# Autodesk Inventor assembly: Ensemble tout
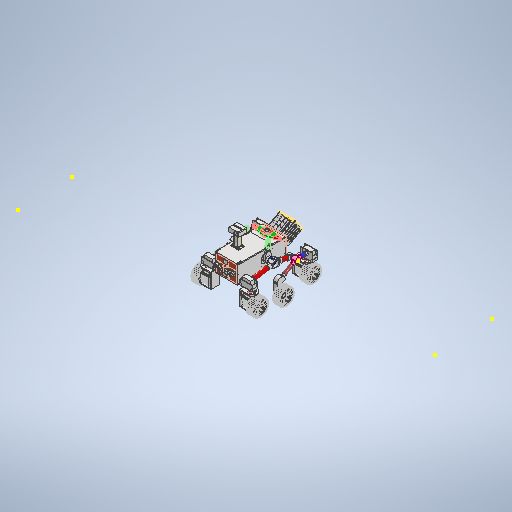
[picture p0: Inventor's stored thumbnail of the model, 512x512]
Saved by Autodesk Inventor 2026.2 (Build 302298010, 298A)
## iProperties
Created: 2026-03-16
Part Number: Ensemble tout
Document SubType Name: Assembly
Designer: genon
Author: genon
## Documents named in this file (36)
- C:\Users\genon\Documents\Henallux Passerelle\Projet de conception\Cassini T-X\Inventor\Ensemble tout.iam
- C:\Users\genon\Documents\Henallux Passerelle\Projet de conception\Cassini T-X\Inventor\Ensemble_Boite_chassis.iam
- C:\Users\genon\Documents\Henallux Passerelle\Projet de conception\Cassini T-X\Inventor\Suspension\Ensemble_Relier_suspension.iam
- C:\Users\genon\Documents\Henallux Passerelle\Projet de conception\Cassini T-X\Inventor\Suspension\tube vers bogie.ipt
- C:\Users\genon\Documents\Henallux Passerelle\Projet de conception\Cassini T-X\Inventor\Suspension\bielle sup.ipt
- C:\Users\genon\Documents\Henallux Passerelle\Projet de conception\Cassini T-X\Inventor\Suspension\bielle côté 0.ipt
- C:\Users\genon\Documents\Henallux Passerelle\Projet de conception\Cassini T-X\Inventor\Suspension\bièlle côté.ipt
- C:\Users\genon\Documents\Henallux Passerelle\Projet de conception\Cassini T-X\Inventor\Suspension\Rolling v2.ipt
- C:\Users\genon\Documents\Henallux Passerelle\Projet de conception\Cassini T-X\Inventor\Suspension\bielle côté 2.ipt
- C:\Users\genon\Documents\Henallux Passerelle\Projet de conception\Cassini T-X\Inventor\Suspension\bielle côté 3.ipt
- C:\Users\genon\Documents\Henallux Passerelle\Projet de conception\Cassini T-X\Inventor\Suspension\tubelong_rocker.ipt
- C:\Users\genon\Documents\Henallux Passerelle\Projet de conception\Cassini T-X\Inventor\Suspension\Attache servomoteur.ipt
- C:\Users\genon\Documents\Henallux Passerelle\Projet de conception\Cassini T-X\Inventor\Suspension\bielle rocker.ipt
- C:\Users\genon\Documents\Henallux Passerelle\Projet de conception\Cassini T-X\Inventor\Suspension\bielle rocker2.ipt
- C:\Users\genon\Documents\Henallux Passerelle\Projet de conception\Cassini T-X\Inventor\Suspension\tube des bogies.ipt
- C:\Users\genon\Documents\Henallux Passerelle\Projet de conception\Cassini T-X\Inventor\Suspension\Attache servomoteur_bogie.ipt
- C:\Users\genon\Documents\Henallux Passerelle\Projet de conception\Cassini T-X\Inventor\Composants\Stepper Motor\Stepper Motor\Stepper Motor.ipt
- C:\Users\genon\Documents\Henallux Passerelle\Projet de conception\Cassini T-X\Inventor\Suspension\roulement 22mm.ipt
- C:\Users\genon\Documents\Henallux Passerelle\Projet de conception\Cassini T-X\Inventor\Suspension\Roue.ipt
- C:\Users\genon\Documents\Henallux Passerelle\Projet de conception\Cassini T-X\Inventor\Suspension\Roue libre.ipt
- C:\Users\genon\Documents\Henallux Passerelle\Projet de conception\Cassini T-X\Inventor\Suspension\bielle roue milieu autre côté.ipt
- C:\Users\genon\Documents\Henallux Passerelle\Projet de conception\Cassini T-X\Inventor\Composants\US HC-SR04.ipt
- C:\Users\genon\Documents\Henallux Passerelle\Projet de conception\Cassini T-X\Inventor\Composants\TOF - VL6180X Fermion SEN0427.ipt
- C:\Users\genon\Documents\Henallux Passerelle\Projet de conception\Cassini T-X\Inventor\Suspension\tube vers roue libre.ipt
- C:\Users\genon\Documents\Henallux Passerelle\Projet de conception\Cassini T-X\Inventor\Accessoires\Caméra.ipt
- C:\Users\genon\Documents\Henallux Passerelle\Projet de conception\Cassini T-X\Inventor\Accessoires\Bras caméra.ipt
- C:\Users\genon\Documents\Henallux Passerelle\Projet de conception\Cassini T-X\Inventor\Accessoires\autour hélice.ipt
- C:\Users\genon\Documents\Henallux Passerelle\Projet de conception\Cassini T-X\Inventor\Accessoires\Bras hélice.ipt
- C:\Users\genon\Documents\Henallux Passerelle\Projet de conception\Cassini T-X\Inventor\Accessoires\Hélice.ipt
- C:\Users\genon\Documents\Henallux Passerelle\Projet de conception\Cassini T-X\Inventor\Accessoires\autour hélice autre côté.ipt
- C:\Users\genon\Documents\Henallux Passerelle\Projet de conception\Cassini T-X\Inventor\Accessoires\au-dessus hélice.ipt
- C:\Users\genon\Downloads\liaison servomoteus\Servomoteur analogique FS5106B.ipt
- C:\Users\genon\Documents\Henallux Passerelle\Projet de conception\Cassini T-X\Inventor\Suspension\support palonnier test.ipt
- C:\Users\genon\Documents\Henallux Passerelle\Projet de conception\Cassini T-X\Inventor\Suspension\support palonnier test v2.ipt
- C:\Users\genon\Documents\Henallux Passerelle\Projet de conception\Cassini T-X\Inventor\Suspension\palonnier.ipt
- C:\Users\genon\Documents\Henallux Passerelle\Projet de conception\Cassini T-X\Inventor\Suspension\bielle roue milieu autre .ipt
## Components (71 placed, 35 different names)
1. Ensemble_Boite_chassis:1 [sub-assembly] — Placage:15, Placage:16, Placage:63, Placage:64, Placage:138, Placage:139, Placage:160, Placage:177, Placage:245, Placage:246, Placage:255, Placage:279, Placage:280, Placage:281, Placage:282, Placage:283, Placage:284, Placage:285, Placage:286, Placage:287, Placage:288, Placage:289, Placage:290, Placage:327, Placage:328
2. Ensemble_Relier_suspension:1 [sub-assembly] — Placage:245, Placage:246
3. bielle sup:1 — Placage:247, Placage:248
4. bielle côté 0:1 — Placage:15, Placage:16, Cylindrique:2, Placage:19, Placage:138
5. bièlle côté:1 — Cylindrique:1, Placage:18, Placage:19, Placage:20, Placage:21, Placage:22, Cylindrique:3, Placage:247, Placage:248
6. Rolling v2:1 — Cylindrique:1, Placage:18, Cylindrique:2
7. bielle côté 2:1 — Placage:20, Placage:21, Placage:22, Placage:23, Placage:149, Placage:150, Placage:151
8. Rolling v2:2 — Cylindrique:3, Placage:23
9. tubelong_rocker:1 — Placage:30, Placage:31, Placage:152, Placage:153
10. Attache servomoteur:1 — Placage:30, Placage:31, Placage:232, Placage:233, Placage:234, Placage:276
11. tube vers bogie:3 — Placage:37, Placage:38, Placage:154, Placage:155
12. bielle rocker:1 — Placage:37, Placage:38, Cylindrique:9, Placage:97
13. bielle rocker2:1 — Placage:43, Placage:44, Placage:145, Placage:146, Placage:357, Placage:358
14. tube des bogies:1 — Placage:43, Placage:44, Placage:47, Placage:48
15. Attache servomoteur_bogie:1 — Placage:47, Placage:48, Placage:329, Placage:330, Placage:331
16. Stepper Motor:1 — Placage:93, Placage:94, Placage:95, Placage:268, Placage:269, Affleurement:9
17. bièlle côté:2 — Placage:65, Placage:66, Placage:67, Placage:68, Placage:69, Placage:70, Placage:249, Placage:250
18. bielle côté 0:2 — Placage:63, Placage:64, Cylindrique:7, Placage:67, Placage:68, Placage:139
19. roulement 22mm:1 — Placage:65, Placage:66, Cylindrique:7
20. bielle côté 2:2 — Placage:69, Placage:70, Cylindrique:8, Placage:71, Placage:72, Placage:73
21. roulement 22mm:2 — Cylindrique:8, Placage:71
22. bielle côté 3:3 — Placage:72, Placage:73, Placage:74, Placage:75, Placage:78, Placage:79
23. tubelong_rocker:2 — Placage:74, Placage:75, Placage:76, Placage:77
24. Attache servomoteur:2 — Placage:76, Placage:77, Placage:229, Placage:230, Placage:231
25. tube vers bogie:4 — Placage:78, Placage:79, Placage:80, Placage:81
26. bielle rocker:2 — Placage:80, Placage:81, Cylindrique:11, Placage:98
27. roulement 22mm:3 — Cylindrique:11, Placage:98, Placage:296, Placage:297
28. bielle rocker2:2 — Placage:86, Placage:87, Placage:156, Placage:157, Placage:296, Placage:297
29. tube des bogies:4 — Placage:86, Placage:87, Placage:298, Placage:299, Placage:300
30. Attache servomoteur_bogie:2 — Placage:298, Placage:299, Placage:300, Placage:301, Placage:302, Placage:303
31. Roue:1 — Placage:114, Placage:115, Placage:116
32. Roue:2 — Placage:93, Placage:94, Placage:95
33. roulement 22mm:4 — Cylindrique:9, Placage:97, Placage:357, Placage:358
34. Roue libre:1 — Cylindrique:13, Placage:101, Placage:337
35. roulement 22mm:5 — Cylindrique:13, Placage:101, Placage:336
36. Stepper Motor:2 — Placage:117, Placage:118, Placage:119, Placage:263, Placage:264, Affleurement:7
37. Stepper Motor:3 — Placage:123, Placage:124, Placage:125, Placage:266, Placage:267, Affleurement:8
38. Stepper Motor:4 — Placage:114, Placage:115, Placage:116, Placage:270, Placage:271, Affleurement:10, Placage:272
39. Roue libre:2 — Cylindrique:14, Placage:120
40. Roue:3 — Placage:117, Placage:118, Placage:119
41. roulement 22mm:6 — Cylindrique:14, Placage:120, Placage:294, Placage:295
42. Roue:4 — Placage:123, Placage:124, Placage:125
43. bielle sup:2 — Placage:249, Placage:250
44. US HC-SR04:1 — Placage:282, Placage:283, Placage:284
45. US HC-SR04:2 — Placage:279, Placage:280, Placage:281
46. TOF - VL6180X Fermion SEN0427:1 — Placage:285, Placage:286, Placage:287
47. TOF - VL6180X Fermion SEN0427:2 — Placage:288, Placage:289, Placage:290
48. tube vers roue libre:1 — Placage:145, Placage:146, Placage:332, Placage:333, Placage:334
49. bielle côté 3:4 — Placage:149, Placage:150, Placage:151, Placage:152, Placage:153, Placage:154, Placage:155
50. tube vers roue libre:2 — Placage:156, Placage:157, Placage:291, Placage:292, Placage:293
51. Bras caméra:1 — Placage:160, Placage:163, Placage:164, Placage:165, Placage:327, Placage:328
52. Caméra:1 — Placage:163, Placage:164, Placage:165
53. Bras hélice:1 — Placage:172, Placage:173
54. Hélice:1 — Placage:172, Placage:173
55. autour hélice:2 — Placage:177, Placage:180, Placage:255, Placage:259, Placage:260
56. autour hélice autre côté:1 — Placage:258
57. au-dessus hélice:1 — Placage:180, Placage:258, Placage:259, Placage:260
58. Servomoteur analogique FS5106B:1 — Placage:301, Placage:302, Placage:303, Placage:341, Placage:342
59. Servomoteur analogique FS5106B:2 — Placage:329, Placage:330, Placage:331, Placage:355, Placage:356
60. Servomoteur analogique FS5106B:3 — Placage:232, Placage:233, Placage:234, Placage:351
61. Servomoteur analogique FS5106B:4 — Placage:229, Placage:230, Placage:231, Placage:346, Placage:347
62. support palonnier test:1 — Placage:263, Placage:264, Affleurement:7, Placage:343, Placage:344, Placage:345, Placage:347
63. support palonnier test:2 — Placage:266, Placage:267, Affleurement:8, Placage:276, Placage:348, Placage:349, Placage:350
64. support palonnier test v2:1 — Placage:268, Placage:269, Affleurement:9, Placage:352, Placage:353, Placage:354, Placage:356
65. support palonnier test v2:2 — Placage:270, Placage:271, Affleurement:10, Placage:272, Placage:338, Placage:339, Placage:340, Placage:342
66. palonnier:3 — Placage:338, Placage:339, Placage:340, Placage:341
67. palonnier:5 — Placage:343, Placage:344, Placage:345, Placage:346
68. bielle roue milieu autre :1 — Placage:291, Placage:292, Placage:293, Placage:294, Placage:295
69. bielle roue milieu autre côté:1 — Placage:332, Placage:333, Placage:334, Placage:336, Placage:337
70. palonnier:6 — Placage:352, Placage:353, Placage:354, Placage:355
71. palonnier:7 — Placage:348, Placage:349, Placage:350, Placage:351
## Relationships (169: Mate 156, CylindricalJoint 9, Flush 4)
- Placage:15 [Mate]: Ensemble_Boite_chassis:1 ↔ bielle côté 0:1
- Placage:16 [Mate]: Ensemble_Boite_chassis:1 ↔ bielle côté 0:1
- Cylindrique:1: bièlle côté:1 ↔ Rolling v2:1
- Placage:18 [Mate]: bièlle côté:1 ↔ Rolling v2:1
- Cylindrique:2: bielle côté 0:1 ↔ Rolling v2:1
- Placage:19 [Mate]: bielle côté 0:1 ↔ bièlle côté:1
- Placage:20 [Mate]: bièlle côté:1 ↔ bielle côté 2:1
- Placage:21 [Mate]: bièlle côté:1 ↔ bielle côté 2:1
- Placage:22 [Mate]: bièlle côté:1 ↔ bielle côté 2:1
- Cylindrique:3: bièlle côté:1 ↔ Rolling v2:2
- Placage:23 [Mate]: bielle côté 2:1 ↔ Rolling v2:2
- Placage:30 [Mate]: tubelong_rocker:1 ↔ Attache servomoteur:1
- Placage:31 [Mate]: tubelong_rocker:1 ↔ Attache servomoteur:1
- Placage:37 [Mate]: tube vers bogie:3 ↔ bielle rocker:1
- Placage:38 [Mate]: tube vers bogie:3 ↔ bielle rocker:1
- Placage:43 [Mate]: bielle rocker2:1 ↔ tube des bogies:1
- Placage:44 [Mate]: bielle rocker2:1 ↔ tube des bogies:1
- Placage:47 [Mate]: tube des bogies:1 ↔ Attache servomoteur_bogie:1
- Placage:48 [Mate]: tube des bogies:1 ↔ Attache servomoteur_bogie:1
- Placage:63 [Mate]: Ensemble_Boite_chassis:1 ↔ bielle côté 0:2
- Placage:64 [Mate]: Ensemble_Boite_chassis:1 ↔ bielle côté 0:2
- Placage:65 [Mate]: bièlle côté:2 ↔ roulement 22mm:1
- Placage:66 [Mate]: bièlle côté:2 ↔ roulement 22mm:1
- Cylindrique:7: bielle côté 0:2 ↔ roulement 22mm:1
- Placage:67 [Mate]: bièlle côté:2 ↔ bielle côté 0:2
- Placage:68 [Mate]: bièlle côté:2 ↔ bielle côté 0:2
- Placage:69 [Mate]: bièlle côté:2 ↔ bielle côté 2:2
- Placage:70 [Mate]: bièlle côté:2 ↔ bielle côté 2:2
- Cylindrique:8: bielle côté 2:2 ↔ roulement 22mm:2
- Placage:71 [Mate]: bielle côté 2:2 ↔ roulement 22mm:2
- Placage:72 [Mate]: bielle côté 2:2 ↔ bielle côté 3:3
- Placage:73 [Mate]: bielle côté 2:2 ↔ bielle côté 3:3
- Placage:74 [Mate]: bielle côté 3:3 ↔ tubelong_rocker:2
- Placage:75 [Mate]: bielle côté 3:3 ↔ tubelong_rocker:2
- Placage:76 [Mate]: tubelong_rocker:2 ↔ Attache servomoteur:2
- Placage:77 [Mate]: tubelong_rocker:2 ↔ Attache servomoteur:2
- Placage:78 [Mate]: bielle côté 3:3 ↔ tube vers bogie:4
- Placage:79 [Mate]: bielle côté 3:3 ↔ tube vers bogie:4
- Placage:80 [Mate]: tube vers bogie:4 ↔ bielle rocker:2
- Placage:81 [Mate]: tube vers bogie:4 ↔ bielle rocker:2
- Placage:86 [Mate]: bielle rocker2:2 ↔ tube des bogies:4
- Placage:87 [Mate]: bielle rocker2:2 ↔ tube des bogies:4
- Placage:93 [Mate]: Stepper Motor:1 ↔ Roue:2
- Placage:94 [Mate]: Stepper Motor:1 ↔ Roue:2
- Placage:95 [Mate]: Stepper Motor:1 ↔ Roue:2
- Cylindrique:9: bielle rocker:1 ↔ roulement 22mm:4
- Placage:97 [Mate]: bielle rocker:1 ↔ roulement 22mm:4
- Cylindrique:11: bielle rocker:2 ↔ roulement 22mm:3
- Placage:98 [Mate]: bielle rocker:2 ↔ roulement 22mm:3
- Cylindrique:13: Roue libre:1 ↔ roulement 22mm:5
- Placage:101 [Mate]: Roue libre:1 ↔ roulement 22mm:5
- Placage:114 [Mate]: Roue:1 ↔ Stepper Motor:4
- Placage:115 [Mate]: Roue:1 ↔ Stepper Motor:4
- Placage:116 [Mate]: Roue:1 ↔ Stepper Motor:4
- Placage:117 [Mate]: Stepper Motor:2 ↔ Roue:3
- Placage:118 [Mate]: Stepper Motor:2 ↔ Roue:3
- Placage:119 [Mate]: Stepper Motor:2 ↔ Roue:3
- Cylindrique:14: Roue libre:2 ↔ roulement 22mm:6
- Placage:120 [Mate]: Roue libre:2 ↔ roulement 22mm:6
- Placage:123 [Mate]: Stepper Motor:3 ↔ Roue:4
- Placage:124 [Mate]: Stepper Motor:3 ↔ Roue:4
- Placage:125 [Mate]: Stepper Motor:3 ↔ Roue:4
- Placage:138 [Mate]: Ensemble_Boite_chassis:1 ↔ bielle côté 0:1
- Placage:139 [Mate]: Ensemble_Boite_chassis:1 ↔ bielle côté 0:2
- Placage:145 [Mate]: bielle rocker2:1 ↔ tube vers roue libre:1
- Placage:146 [Mate]: bielle rocker2:1 ↔ tube vers roue libre:1
- Placage:149 [Mate]: bielle côté 2:1 ↔ bielle côté 3:4
- Placage:150 [Mate]: bielle côté 2:1 ↔ bielle côté 3:4
- Placage:151 [Mate]: bielle côté 2:1 ↔ bielle côté 3:4
- Placage:152 [Mate]: tubelong_rocker:1 ↔ bielle côté 3:4
- Placage:153 [Mate]: tubelong_rocker:1 ↔ bielle côté 3:4
- Placage:154 [Mate]: tube vers bogie:3 ↔ bielle côté 3:4
- Placage:155 [Mate]: tube vers bogie:3 ↔ bielle côté 3:4
- Placage:156 [Mate]: bielle rocker2:2 ↔ tube vers roue libre:2
- Placage:157 [Mate]: bielle rocker2:2 ↔ tube vers roue libre:2
- Placage:160 [Mate]: Ensemble_Boite_chassis:1 ↔ Bras caméra:1
- Placage:163 [Mate]: Bras caméra:1 ↔ Caméra:1
- Placage:164 [Mate]: Bras caméra:1 ↔ Caméra:1
- Placage:165 [Mate]: Bras caméra:1 ↔ Caméra:1
- Placage:172 [Mate]: Bras hélice:1 ↔ Hélice:1
- Placage:173 [Mate]: Bras hélice:1 ↔ Hélice:1
- Placage:177 [Mate]: Ensemble_Boite_chassis:1 ↔ autour hélice:2
- Placage:180 [Mate]: autour hélice:2 ↔ au-dessus hélice:1
- Placage:229 [Mate]: Attache servomoteur:2 ↔ Servomoteur analogique FS5106B:4
- Placage:230 [Mate]: Attache servomoteur:2 ↔ Servomoteur analogique FS5106B:4
- Placage:231 [Mate]: Attache servomoteur:2 ↔ Servomoteur analogique FS5106B:4
- Placage:232 [Mate]: Attache servomoteur:1 ↔ Servomoteur analogique FS5106B:3
- Placage:233 [Mate]: Attache servomoteur:1 ↔ Servomoteur analogique FS5106B:3
- Placage:234 [Mate]: Attache servomoteur:1 ↔ Servomoteur analogique FS5106B:3
- Placage:245 [Mate]: Ensemble_Boite_chassis:1 ↔ Ensemble_Relier_suspension:1
- Placage:246 [Mate]: Ensemble_Boite_chassis:1 ↔ Ensemble_Relier_suspension:1
- Placage:247 [Mate]: bielle sup:1 ↔ bièlle côté:1
- Placage:248 [Mate] (0.4 mm): bielle sup:1 ↔ bièlle côté:1
- Placage:249 [Mate]: bièlle côté:2 ↔ bielle sup:2
- Placage:250 [Mate] (0.4 mm): bièlle côté:2 ↔ bielle sup:2
- Placage:255 [Mate]: Ensemble_Boite_chassis:1 ↔ autour hélice:2
- Placage:258 [Mate]: autour hélice autre côté:1 ↔ au-dessus hélice:1
- Placage:259 [Mate]: autour hélice:2 ↔ au-dessus hélice:1
- Placage:260 [Mate]: autour hélice:2 ↔ au-dessus hélice:1
- Placage:263 [Mate]: Stepper Motor:2 ↔ support palonnier test:1
- Placage:264 [Mate]: Stepper Motor:2 ↔ support palonnier test:1
- Affleurement:7 [Flush] (2.2 mm): Stepper Motor:2 ↔ support palonnier test:1
- Placage:266 [Mate]: Stepper Motor:3 ↔ support palonnier test:2
- Placage:267 [Mate]: Stepper Motor:3 ↔ support palonnier test:2
- Affleurement:8 [Flush] (2 mm): Stepper Motor:3 ↔ support palonnier test:2
- Placage:268 [Mate]: Stepper Motor:1 ↔ support palonnier test v2:1
- Placage:269 [Mate]: Stepper Motor:1 ↔ support palonnier test v2:1
- Affleurement:9 [Flush] (2 mm): Stepper Motor:1 ↔ support palonnier test v2:1
- Placage:270 [Mate]: Stepper Motor:4 ↔ support palonnier test v2:2
- Placage:271 [Mate]: Stepper Motor:4 ↔ support palonnier test v2:2
- Affleurement:10 [Flush] (2 mm): Stepper Motor:4 ↔ support palonnier test v2:2
- Placage:272 [Mate]: Stepper Motor:4 ↔ support palonnier test v2:2
- Placage:276 [Mate] (5 mm): Attache servomoteur:1 ↔ support palonnier test:2
- Placage:279 [Mate]: Ensemble_Boite_chassis:1 ↔ US HC-SR04:2
- Placage:280 [Mate] (-2 mm): Ensemble_Boite_chassis:1 ↔ US HC-SR04:2
- Placage:281 [Mate] (-3 mm): Ensemble_Boite_chassis:1 ↔ US HC-SR04:2
- Placage:282 [Mate]: Ensemble_Boite_chassis:1 ↔ US HC-SR04:1
- Placage:283 [Mate] (-2 mm): Ensemble_Boite_chassis:1 ↔ US HC-SR04:1
- Placage:284 [Mate] (-3 mm): Ensemble_Boite_chassis:1 ↔ US HC-SR04:1
- Placage:285 [Mate]: Ensemble_Boite_chassis:1 ↔ TOF - VL6180X Fermion SEN0427:1
- Placage:286 [Mate]: Ensemble_Boite_chassis:1 ↔ TOF - VL6180X Fermion SEN0427:1
- Placage:287 [Mate]: Ensemble_Boite_chassis:1 ↔ TOF - VL6180X Fermion SEN0427:1
- Placage:288 [Mate]: Ensemble_Boite_chassis:1 ↔ TOF - VL6180X Fermion SEN0427:2
- Placage:289 [Mate]: Ensemble_Boite_chassis:1 ↔ TOF - VL6180X Fermion SEN0427:2
- Placage:290 [Mate]: Ensemble_Boite_chassis:1 ↔ TOF - VL6180X Fermion SEN0427:2
- Placage:291 [Mate]: tube vers roue libre:2 ↔ bielle roue milieu autre :1
- Placage:292 [Mate]: tube vers roue libre:2 ↔ bielle roue milieu autre :1
- Placage:293 [Mate]: tube vers roue libre:2 ↔ bielle roue milieu autre :1
- Placage:294 [Mate]: roulement 22mm:6 ↔ bielle roue milieu autre :1
- Placage:295 [Mate]: roulement 22mm:6 ↔ bielle roue milieu autre :1
- Placage:296 [Mate]: roulement 22mm:3 ↔ bielle rocker2:2
- Placage:297 [Mate]: roulement 22mm:3 ↔ bielle rocker2:2
- Placage:298 [Mate]: tube des bogies:4 ↔ Attache servomoteur_bogie:2
- Placage:299 [Mate]: tube des bogies:4 ↔ Attache servomoteur_bogie:2
- Placage:300 [Mate]: tube des bogies:4 ↔ Attache servomoteur_bogie:2
- Placage:301 [Mate]: Attache servomoteur_bogie:2 ↔ Servomoteur analogique FS5106B:1
- Placage:302 [Mate]: Attache servomoteur_bogie:2 ↔ Servomoteur analogique FS5106B:1
- Placage:303 [Mate]: Attache servomoteur_bogie:2 ↔ Servomoteur analogique FS5106B:1
- Placage:327 [Mate]: Ensemble_Boite_chassis:1 ↔ Bras caméra:1
- Placage:328 [Mate]: Ensemble_Boite_chassis:1 ↔ Bras caméra:1
- Placage:329 [Mate]: Attache servomoteur_bogie:1 ↔ Servomoteur analogique FS5106B:2
- Placage:330 [Mate]: Attache servomoteur_bogie:1 ↔ Servomoteur analogique FS5106B:2
- Placage:331 [Mate]: Attache servomoteur_bogie:1 ↔ Servomoteur analogique FS5106B:2
- Placage:332 [Mate]: tube vers roue libre:1 ↔ bielle roue milieu autre côté:1
- Placage:333 [Mate]: tube vers roue libre:1 ↔ bielle roue milieu autre côté:1
- Placage:334 [Mate]: tube vers roue libre:1 ↔ bielle roue milieu autre côté:1
- Placage:336 [Mate]: roulement 22mm:5 ↔ bielle roue milieu autre côté:1
- Placage:337 [Mate]: Roue libre:1 ↔ bielle roue milieu autre côté:1
- Placage:338 [Mate]: support palonnier test v2:2 ↔ palonnier:3
- Placage:339 [Mate] (2.5 mm): support palonnier test v2:2 ↔ palonnier:3
- Placage:340 [Mate] (3 mm): support palonnier test v2:2 ↔ palonnier:3
- Placage:341 [Mate]: Servomoteur analogique FS5106B:1 ↔ palonnier:3
- Placage:342 [Mate]: Servomoteur analogique FS5106B:1 ↔ support palonnier test v2:2
- Placage:343 [Mate]: support palonnier test:1 ↔ palonnier:5
- Placage:344 [Mate] (2.5 mm): support palonnier test:1 ↔ palonnier:5
- Placage:345 [Mate] (2 mm): support palonnier test:1 ↔ palonnier:5
- Placage:346 [Mate]: Servomoteur analogique FS5106B:4 ↔ palonnier:5
- Placage:347 [Mate]: Servomoteur analogique FS5106B:4 ↔ support palonnier test:1
- Placage:348 [Mate]: support palonnier test:2 ↔ palonnier:7
- Placage:349 [Mate] (2 mm): support palonnier test:2 ↔ palonnier:7
- Placage:350 [Mate] (3 mm): support palonnier test:2 ↔ palonnier:7
- Placage:351 [Mate]: Servomoteur analogique FS5106B:3 ↔ palonnier:7
- Placage:352 [Mate]: support palonnier test v2:1 ↔ palonnier:6
- Placage:353 [Mate] (2 mm): support palonnier test v2:1 ↔ palonnier:6
- Placage:354 [Mate] (3 mm): support palonnier test v2:1 ↔ palonnier:6
- Placage:355 [Mate]: Servomoteur analogique FS5106B:2 ↔ palonnier:6
- Placage:356 [Mate]: Servomoteur analogique FS5106B:2 ↔ support palonnier test v2:1
- Placage:357 [Mate]: bielle rocker2:1 ↔ roulement 22mm:4
- Placage:358 [Mate]: bielle rocker2:1 ↔ roulement 22mm:4
